# Autodesk Inventor assembly: Hexagonal with LEDs Assembly
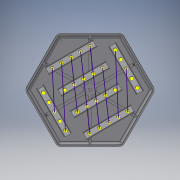
[picture p0: Inventor's stored thumbnail of the model, 180x180]
Saved by Autodesk Inventor 2019 (Build 230136000, 136)
## iProperties
Created: 2022-03-28
Part Number: Hexagonal with LEDs Assembly
Document SubType Name: Assembly
Designer: Lix
Author: Lix
## Documents named in this file (3)
- G:\Project\Hybrids\HexaWall\Inventor\Hexagonal with LEDs Assembly.iam
- G:\Project\Hybrids\HexaWall\Inventor\Base v6 - 175 - thicker wall.ipt
- G:\Project\Hybrids\HexaWall\Inventor\LED Strip 5050 x 5.ipt
## Components (7 placed, 2 different names)
1. Base v6 - 175 - thicker wall:1 — Mate:1, Mate:2, Flush:1, Mate:3, Flush:2, Mate:4, Mate:5, Mate:6, Mate:7, Mate:8, Flush:3, Mate:9, Flush:4
2. LED Strip 5050 x 5:1 — Mate:1, Mate:2, Flush:1
3. LED Strip 5050 x 5:2 — Mate:3, Flush:2, Mate:4
4. LED Strip 5050 x 5:3 — Mate:8, Flush:3, Mate:9
5. LED Strip 5050 x 5:4
6. LED Strip 5050 x 5:5
7. LED Strip 5050 x 5:6
## Component patterns: (4 elements, first: LED Strip 5050 x 5:3)
## Relationships (13: Mate 9, Flush 4)
- Mate:1: Base v6 - 175 - thicker wall:1 ↔ LED Strip 5050 x 5:1
- Mate:2 (0.5 mm): Base v6 - 175 - thicker wall:1 ↔ LED Strip 5050 x 5:1
- Flush:1 (0.8 mm): Base v6 - 175 - thicker wall:1 ↔ LED Strip 5050 x 5:1
- Mate:3 (0.5 mm): Base v6 - 175 - thicker wall:1 ↔ LED Strip 5050 x 5:2
- Flush:2 (0.8 mm): Base v6 - 175 - thicker wall:1 ↔ LED Strip 5050 x 5:2
- Mate:4: Base v6 - 175 - thicker wall:1 ↔ LED Strip 5050 x 5:2
- Mate:5: Base v6 - 175 - thicker wall:1
- Mate:6: Base v6 - 175 - thicker wall:1
- Mate:7 (-1.5 mm): Base v6 - 175 - thicker wall:1
- Mate:8 (0.5 mm): Base v6 - 175 - thicker wall:1 ↔ LED Strip 5050 x 5:3
- Flush:3 (0.8 mm): Base v6 - 175 - thicker wall:1 ↔ LED Strip 5050 x 5:3
- Mate:9: Base v6 - 175 - thicker wall:1 ↔ LED Strip 5050 x 5:3
- Flush:4 (10 mm): Base v6 - 175 - thicker wall:1
